# Autodesk Inventor assembly: Assembly1
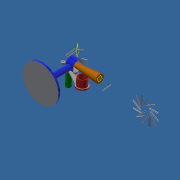
[picture p0: Inventor's stored thumbnail of the model, 180x180]
Saved by Autodesk Inventor 2018 (Build 220112000, 112)
## iProperties
Created: 2022-02-21
Part Number: Assembly1
Document SubType Name: Assembly
Designer: Nathann
Author: Nathann
## Documents named in this file (9)
- C:\Users\Nathann\OneDrive\Objet3D\EPFLEplucheCarrote\Assembly1.iam
- C:\Users\Nathann\OneDrive\Objet3D\EPFLEplucheCarrote\Feet.ipt
- C:\Users\Nathann\OneDrive\Objet3D\EPFLEplucheCarrote\Manivelle.ipt
- C:\Users\Nathann\OneDrive\Objet3D\EPFLEplucheCarrote\Handle.ipt
- C:\Users\Nathann\OneDrive\Objet3D\EPFLEplucheCarrote\Carrote.ipt
- C:\Users\Nathann\OneDrive\Objet3D\EPFLEplucheCarrote\Carrot_Peeler_Blade.ipt
- C:\Users\Nathann\OneDrive\Objet3D\FaucetLaminarFlow\CarrotRoller.ipt
- C:\Users\Nathann\OneDrive\Objet3D\FaucetLaminarFlow\SpringLoadedRollerHolder.ipt
- C:\Users\Nathann\OneDrive\Objet3D\FaucetLaminarFlow\BladeHolderSpringLoaded.ipt
## Components (23 placed, 8 different names)
1. Feet:1 — Mate:2, Mate:5, Mate:6
2. Manivelle:1 — Flush:2
3. Handle:1 — Flush:2
4. Carrote:1 — Mate:2
5. Carrot_Peeler_Blade:1 — Mate:3, Insert:2, Flush:3
6. CarrotRoller:1
7. SpringLoadedRollerHolder:1 — Mate:5
8. BladeHolderSpringLoaded:1 — Mate:3, Insert:2, Flush:3, Mate:4, Angle:1, Flush:4, Mate:6
9. Carrot_Peeler_Blade:3
10. Carrot_Peeler_Blade:4
11. CarrotRoller:2
12. Carrot_Peeler_Blade:2
13. Carrot_Peeler_Blade:5
14. Carrot_Peeler_Blade:6
15. Carrot_Peeler_Blade:7
16. Carrot_Peeler_Blade:8
17. Carrot_Peeler_Blade:9
18. Carrot_Peeler_Blade:10
19. Carrot_Peeler_Blade:11
20. Carrot_Peeler_Blade:12
21. Carrot_Peeler_Blade:13
22. Carrot_Peeler_Blade:14
23. Carrot_Peeler_Blade:15
## Component patterns: (12 elements, first: Carrot_Peeler_Blade:2)
## Relationships (10: Mate 5, Flush 3, Insert 1, Angle 1)
- Flush:2: Manivelle:1 ↔ Handle:1
- Mate:2: Feet:1 ↔ Carrote:1
- Mate:3: Carrot_Peeler_Blade:1 ↔ BladeHolderSpringLoaded:1
- Insert:2: Carrot_Peeler_Blade:1 ↔ BladeHolderSpringLoaded:1
- Flush:3: Carrot_Peeler_Blade:1 ↔ BladeHolderSpringLoaded:1
- Mate:4: BladeHolderSpringLoaded:1
- Angle:1 (45 deg): BladeHolderSpringLoaded:1
- Flush:4: BladeHolderSpringLoaded:1
- Mate:5: Feet:1 ↔ SpringLoadedRollerHolder:1
- Mate:6: Feet:1 ↔ BladeHolderSpringLoaded:1
